# Autodesk Inventor assembly: ASSEMBLY_Main
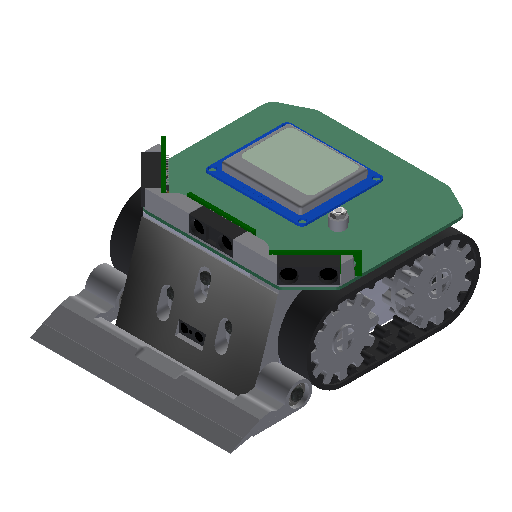
[picture p0: Inventor's stored thumbnail of the model, 512x512]
Saved by Autodesk Inventor 2026.1 (Build 301233000, 233)
## iProperties
Created: 2016-04-29
Part Number: ASSEMBLY_Main
Material: Ogólny
Document SubType Name: Assembly
Designer: Andrzej
Mass: 284.983 g
Surface Area: 1623.62 cm^2
Volume: 252.585 cm^3
Density: 1.12827 g/cm^3
Author: Andrzej
## Documents named in this file (32)
- C:\Users\Andrzej\OneDrive\_DRIVE_SYNCH_FILES\__ BYTECHLAB PROJECTS\MLTDIS - Mini Sumo Robot - Bullet XT\MCAD\1_REV1\ASSEMBLY_MAIN_REVA\ASSEMBLY_Main.iam
- C:\Users\Andrzej\OneDrive\_DRIVE_SYNCH_FILES\__ BYTECHLAB PROJECTS\MLTDIS - Mini Sumo Robot - Bullet XT\MCAD\1_REV1\__COTS_PARTS\COTS_POLOLU_24Dx48L_HP.ipt
- C:\Users\Andrzej\OneDrive\_DRIVE_SYNCH_FILES\__ BYTECHLAB PROJECTS\MLTDIS - Mini Sumo Robot - Bullet XT\MCAD\1_REV1\ASSEMBLY_MAIN_REVA\3DP_PLA_Main_frame.ipt
- C:\Users\Andrzej\OneDrive\_DRIVE_SYNCH_FILES\__ BYTECHLAB PROJECTS\MLTDIS - Mini Sumo Robot - Bullet XT\MCAD\1_REV1\__COTS_PARTS\COTS_AST_604HZZ_Bearing.ipt
- C:\Users\Andrzej\OneDrive\_DRIVE_SYNCH_FILES\__ BYTECHLAB PROJECTS\MLTDIS - Mini Sumo Robot - Bullet XT\MCAD\1_REV1\ASSEMBLY_MAIN_REVA\3DP_PLA_Motor_mounting_bracket_front.ipt
- C:\Users\Andrzej\OneDrive\_DRIVE_SYNCH_FILES\__ BYTECHLAB PROJECTS\MLTDIS - Mini Sumo Robot - Bullet XT\MCAD\1_REV1\__COTS_PARTS\COTS_GENERIC_LiPo_Baterry.ipt
- C:\Users\Andrzej\OneDrive\_DRIVE_SYNCH_FILES\__ BYTECHLAB PROJECTS\MLTDIS - Mini Sumo Robot - Bullet XT\MCAD\1_REV1\__COTS_PARTS\COTS_SHARP_GP2Y0D810Z0F_sensor.ipt
- C:\Users\Andrzej\OneDrive\_DRIVE_SYNCH_FILES\__ BYTECHLAB PROJECTS\MLTDIS - Mini Sumo Robot - Bullet XT\MCAD\1_REV1\ASSEMBLY_MAIN_REVA\3DP_PLA_Front_plow.ipt
- C:\Users\Andrzej\OneDrive\_DRIVE_SYNCH_FILES\__ BYTECHLAB PROJECTS\MLTDIS - Mini Sumo Robot - Bullet XT\MCAD\1_REV1\ASSEMBLY_MAIN_REVA\3DP_PLA_Motor_mounting_bracket_back.ipt
- C:\Users\Andrzej\OneDrive\_DRIVE_SYNCH_FILES\__ BYTECHLAB PROJECTS\MLTDIS - Mini Sumo Robot - Bullet XT\MCAD\1_REV1\__COTS_PARTS\COTS_Nokia_5110_LCD_display.ipt
- C:\Users\Andrzej\OneDrive\_DRIVE_SYNCH_FILES\__ BYTECHLAB PROJECTS\MLTDIS - Mini Sumo Robot - Bullet XT\MCAD\1_REV1\ASSEMBLY_MAIN_REVA\3DP_PLA_Front_motor_clamp_hole_plug.ipt
- C:\Users\Andrzej\OneDrive\_DRIVE_SYNCH_FILES\__ BYTECHLAB PROJECTS\MLTDIS - Mini Sumo Robot - Bullet XT\MCAD\1_REV1\ASSEMBLY_MAIN_REVA\3DP_PLA_Back_motor_clamp_hole_plug.ipt
- C:\Users\Andrzej\OneDrive\_DRIVE_SYNCH_FILES\__ BYTECHLAB PROJECTS\MLTDIS - Mini Sumo Robot - Bullet XT\MCAD\1_REV1\ASSEMBLY_MAIN_REVA\3DP_PLA_Back_slider.ipt
- C:\Users\Andrzej\OneDrive\_DRIVE_SYNCH_FILES\__ BYTECHLAB PROJECTS\MLTDIS - Mini Sumo Robot - Bullet XT\MCAD\1_REV1\ASSEMBLY_MAIN_REVA\ASSEMBLY_PCB_Line_sensor.ipt
- C:\Users\Andrzej\OneDrive\_DRIVE_SYNCH_FILES\__ BYTECHLAB PROJECTS\MLTDIS - Mini Sumo Robot - Bullet XT\MCAD\1_REV1\ASSEMBLY_MAIN_REVA\ASSEMBLY_PCB_Line_sensor_mir.ipt
- C:\Users\Andrzej\OneDrive\_DRIVE_SYNCH_FILES\__ BYTECHLAB PROJECTS\MLTDIS - Mini Sumo Robot - Bullet XT\MCAD\1_REV1\__COTS_PARTS\COTS_SHARP_GP2Y0D810Z0F_sensor_no_pcb.ipt
- C:\Users\Andrzej\OneDrive\_DRIVE_SYNCH_FILES\__ BYTECHLAB PROJECTS\MLTDIS - Mini Sumo Robot - Bullet XT\MCAD\1_REV1\ASSEMBLY_MAIN_REVA\ASSEMBLY_Blade.iam
- C:\Users\Andrzej\OneDrive\_DRIVE_SYNCH_FILES\__ BYTECHLAB PROJECTS\MLTDIS - Mini Sumo Robot - Bullet XT\MCAD\1_REV1\ASSEMBLY_MAIN_REVA\ASSEMBLY_PCB_Motherboard.ipt
- C:\Users\Andrzej\OneDrive\_DRIVE_SYNCH_FILES\__ BYTECHLAB PROJECTS\MLTDIS - Mini Sumo Robot - Bullet XT\MCAD\1_REV1\ASSEMBLY_MAIN_REVA\ASSEMBLY_Tracks.iam
- C:\Users\Andrzej\OneDrive\_DRIVE_SYNCH_FILES\__ BYTECHLAB PROJECTS\MLTDIS - Mini Sumo Robot - Bullet XT\MCAD\1_REV1\__CONTENT_CENTER_PARTS\en-US\ISO 7380-1\ISO 7380-1 - M4 x 25.ipt
- C:\Users\Andrzej\OneDrive\_DRIVE_SYNCH_FILES\__ BYTECHLAB PROJECTS\MLTDIS - Mini Sumo Robot - Bullet XT\MCAD\1_REV1\__CONTENT_CENTER_PARTS\en-US\DIN 125-2  A\DIN 125-2 - A 4,3A.ipt
- C:\Users\Andrzej\OneDrive\_DRIVE_SYNCH_FILES\__ BYTECHLAB PROJECTS\MLTDIS - Mini Sumo Robot - Bullet XT\MCAD\1_REV1\__CONTENT_CENTER_PARTS\en-US\DIN 934\DIN 934 - M4 x 0,7.ipt
- C:\Users\Andrzej\OneDrive\_DRIVE_SYNCH_FILES\__ BYTECHLAB PROJECTS\MLTDIS - Mini Sumo Robot - Bullet XT\MCAD\1_REV1\ASSEMBLY_MAIN_REVA\3DP_PLA_Wheel_cover.ipt
- C:\Users\Andrzej\OneDrive\_DRIVE_SYNCH_FILES\__ BYTECHLAB PROJECTS\MLTDIS - Mini Sumo Robot - Bullet XT\MCAD\1_REV1\__CONTENT_CENTER_PARTS\en-US\ISO 7380-1\ISO 7380-1 - M3 x 30.ipt
- C:\Users\Andrzej\OneDrive\_DRIVE_SYNCH_FILES\__ BYTECHLAB PROJECTS\MLTDIS - Mini Sumo Robot - Bullet XT\MCAD\1_REV1\__CONTENT_CENTER_PARTS\en-US\DIN 934\DIN 934 - M3 x 0,5.ipt
- C:\Users\Andrzej\OneDrive\_DRIVE_SYNCH_FILES\__ BYTECHLAB PROJECTS\MLTDIS - Mini Sumo Robot - Bullet XT\MCAD\1_REV1\__CONTENT_CENTER_PARTS\en-US\DIN 125-2  A\DIN 125-2 - A 3,2A.ipt
- C:\Users\Andrzej\OneDrive\_DRIVE_SYNCH_FILES\__ BYTECHLAB PROJECTS\MLTDIS - Mini Sumo Robot - Bullet XT\MCAD\1_REV1\__CONTENT_CENTER_PARTS\en-US\ISO 7380-1\ISO 7380-1 - M3 x 8.ipt
- C:\Users\Andrzej\OneDrive\_DRIVE_SYNCH_FILES\__ BYTECHLAB PROJECTS\MLTDIS - Mini Sumo Robot - Bullet XT\MCAD\1_REV1\__CONTENT_CENTER_PARTS\en-US\ISO 7380-1\ISO 7380-1 - M3 x 10.ipt
- C:\Users\Andrzej\OneDrive\_DRIVE_SYNCH_FILES\__ BYTECHLAB PROJECTS\MLTDIS - Mini Sumo Robot - Bullet XT\MCAD\1_REV1\__CONTENT_CENTER_PARTS\en-US\ISO 7380-1\ISO 7380-1 - M3 x 25.ipt
- C:\Users\Andrzej\OneDrive\_DRIVE_SYNCH_FILES\__ BYTECHLAB PROJECTS\MLTDIS - Mini Sumo Robot - Bullet XT\MCAD\1_REV1\ASSEMBLY_MAIN_REVA\CUT_M3_Threaded_rod.ipt
- C:\Users\Andrzej\OneDrive\_DRIVE_SYNCH_FILES\__ BYTECHLAB PROJECTS\MLTDIS - Mini Sumo Robot - Bullet XT\MCAD\1_REV1\ASSEMBLY_MAIN_REVA\3DP_PLA_Front_Sharp_sensors_mounting_bracket.ipt
- C:\Users\Andrzej\OneDrive\_DRIVE_SYNCH_FILES\__ BYTECHLAB PROJECTS\MLTDIS - Mini Sumo Robot - Bullet XT\MCAD\1_REV1\ASSEMBLY_MAIN_REVA\3DP_PLA_M3_screw_washer.ipt
## Components (103 placed, 31 different names)
1. COTS_POLOLU_24Dx48L_HP:1 — Równoległy:3, Styczny:7, Styczny:8, Mate:96
2. COTS_POLOLU_24Dx48L_HP:2 — Styczny:1, Równoległy:2, Mate:99
3. 3DP_PLA_Main_frame:1 — Styczny:1, Równoległy:2, Zestawiający:2, Styczny:2, Zestawiający:3, Styczny:3, Zestawiający:4, Styczny:4, Zestawiający:5, Styczny:5, Równoległy:3, Styczny:7, Zestawiający:8, Równoległy:4, Zestawiający:18, Zestawiający:19, Zestawiający:20, Zestawiający:21, Zestawiający:22, Równoległy:6, Równoległy:7, Równoległy:10, Zestawiający:27, Zestawiający:28, Równoległy:11, Równoległy:12, Zestawiający:59, Równoległy:13, Zestawiający:60, Równoległy:14, Równoległy:15, Zestawiający:79, Zestawiający:82, Mate:95, Flush:19, Flush:20, Angle:1, Mate:123, Mate:134, Mate:136, Mate:138, Mate:139, Mate:140, Mate:142, Mate:144, Mate:146, Mate:148, Mate:149, Mate:151, Mate:152, Mate:153, Mate:155, Mate:157, Mate:158, Mate:159, Mate:160, Mate:165, Mate:166, Mate:167, Mate:168
4. COTS_AST_604HZZ_Bearing:1 — Zestawiający:3, Styczny:3, Mate:108
5. COTS_AST_604HZZ_Bearing:2 — Zestawiający:4, Styczny:4, Mate:104
6. COTS_AST_604HZZ_Bearing:3 — Zestawiający:5, Styczny:5, Mate:100
7. COTS_AST_604HZZ_Bearing:4 — Zestawiający:2, Styczny:2, Mate:97, Mate:98
8. 3DP_PLA_Motor_mounting_bracket_front:2 — Zestawiający:8, Styczny:8, Równoległy:4, Zestawiający:57, Mate:125, Mate:127, Mate:129, Mate:131, Mate:141, Mate:143, Mate:145, Mate:147
9. COTS_SHARP_GP2Y0D810Z0F_sensor:1 — Mate:172, Mate:173
10. COTS_SHARP_GP2Y0D810Z0F_sensor:2 — Mate:170, Mate:175
11. COTS_SHARP_GP2Y0D810Z0F_sensor:3 — Mate:171, Mate:174, Mate:176
12. COTS_GENERIC_LiPo_Baterry:1 — Zestawiający:18, Zestawiający:19
13. COTS_GENERIC_LiPo_Baterry:2 — Zestawiający:20, Zestawiający:21
14. 3DP_PLA_Front_plow:1 — Zestawiający:22, Równoległy:6, Równoległy:7, Zestawiający:61, Zestawiający:62, Zestawiający:63, Zestawiający:64, Zestawiający:65, Zestawiający:66, Zestawiający:78, Zestawiający:85, Równoległy:18, Zestawiający:94, Styczny:12, Mate:150, Mate:154, Mate:156
15. 3DP_PLA_Motor_mounting_bracket_back:1 — Równoległy:10, Zestawiający:27, Zestawiający:28, Zestawiający:58, Mate:117, Mate:118, Mate:119, Mate:120, Mate:121, Mate:122, Mate:124, Mate:126, Mate:128, Mate:130, Mate:132, Mate:133, Mate:135, Mate:137
16. COTS_Nokia_5110_LCD_display:1 — Mate:181
17. 3DP_PLA_Front_motor_clamp_hole_plug:1 — Zestawiający:57, Równoległy:11, Równoległy:12
18. 3DP_PLA_Back_motor_clamp_hole_plug:1 — Zestawiający:58, Zestawiający:59, Równoległy:13
19. 3DP_PLA_Back_slider:1 — Zestawiający:60, Równoległy:14, Równoległy:15, Zestawiający:80, Zestawiający:81, Zestawiający:83, Zestawiający:84
20. ASSEMBLY_PCB_Line_sensor:1 — Zestawiający:61, Zestawiający:62, Zestawiający:63
21. ASSEMBLY_PCB_Line_sensor_mir:1 — Zestawiający:64, Zestawiający:65, Zestawiający:66
22. COTS_SHARP_GP2Y0D810Z0F_sensor_no_pcb:1 — Zestawiający:78, Zestawiający:85, Równoległy:18
23. ASSEMBLY_PCB_Line_sensor_mir:2 — Zestawiający:79, Zestawiający:80, Zestawiający:81
24. ASSEMBLY_PCB_Line_sensor:2 — Zestawiający:82, Zestawiający:83, Zestawiający:84
25. ASSEMBLY_Blade:1 [sub-assembly] — Zestawiający:94, Styczny:12, Mate:161, Mate:162, Mate:163, Mate:164
26. ASSEMBLY_PCB_Motherboard:1 — Mate:95, Flush:19, Flush:20, Mate:169, Flush:21, Flush:22, Mate:177, Mate:178, Mate:181
27. ASSEMBLY_Tracks:1 [sub-assembly] — Mate:99, Mate:100, Angle:1, Mate:105, Mate:106, Mate:107, Mate:109, Mate:110, Mate:111, Mate:112
28. ASSEMBLY_Tracks:2 [sub-assembly] — Mate:96, Mate:97, Mate:98, Mate:101, Mate:102, Mate:103, Mate:113, Mate:114, Mate:115, Mate:116
29. 3DP_PLA_Wheel_cover:1 — Mate:110, Mate:111
30. 3DP_PLA_Wheel_cover:2 — Mate:109, Mate:112
31. 3DP_PLA_Wheel_cover:3 — Mate:113, Mate:116
32. 3DP_PLA_Wheel_cover:4 — Mate:114, Mate:115
33. 3DP_PLA_Front_Sharp_sensors_mounting_bracket:1 — Mate:169, Flush:21, Flush:22, Mate:170, Mate:171, Mate:172, Mate:173, Mate:174, Mate:175, Mate:176
34. 3DP_PLA_M3_screw_washer:1 — Mate:177, Mate:180, Insert:38
35. 3DP_PLA_M3_screw_washer:2 — Mate:178, Mate:179, Insert:37
36. ISO 7380-1 M4 x 25:1 — Mate:101, Mate:102
37. DIN 125-2 A A 4,3:1 — Mate:103, Mate:104, Insert:1
38. DIN 934 - replaced by DIN EN 24032/28673/28674 M4:1 — Insert:1
39. ISO 7380-1 M4 x 25:2 — Mate:105, Mate:106
40. DIN 125-2 A A 4,3:2 — Mate:107, Mate:108, Insert:2
41. DIN 934 - replaced by DIN EN 24032/28673/28674 M4:2 — Insert:2
42. DIN 934 - replaced by DIN EN 24032/28673/28674 M3:12 — Insert:37
43. DIN 934 - replaced by DIN EN 24032/28673/28674 M3:13 — Insert:38
44. CUT_M3_Threaded_rod:2 — Mate:166, Mate:168, Mate:180
45. CUT_M3_Threaded_rod:1 — Mate:165, Mate:167, Mate:179
46. ISO 7380-1 M3 x 25:2 — Insert:36
47. DIN 125-2 A A 3,2:34 — Mate:163, Mate:164, Insert:36
48. ISO 7380-1 M3 x 25:1 — Insert:35
49. DIN 125-2 A A 3,2:33 — Mate:161, Mate:162, Insert:35
50. DIN 934 - replaced by DIN EN 24032/28673/28674 M3:11 — Mate:159, Mate:160
51. ISO 7380-1 M3 x 10:2 — Mate:155, Mate:156
52. DIN 934 - replaced by DIN EN 24032/28673/28674 M3:10 — Mate:157, Mate:158
53. ISO 7380-1 M3 x 10:1 — Mate:153, Mate:154
54. DIN 934 - replaced by DIN EN 24032/28673/28674 M3:9 — Mate:151, Mate:152
55. ISO 7380-1 M3 x 8:1 — Mate:149, Mate:150
56. DIN 934 - replaced by DIN EN 24032/28673/28674 M3:8 — Mate:147, Mate:148
57. DIN 934 - replaced by DIN EN 24032/28673/28674 M3:7 — Mate:145, Mate:146
58. DIN 934 - replaced by DIN EN 24032/28673/28674 M3:6 — Mate:143, Mate:144
59. DIN 934 - replaced by DIN EN 24032/28673/28674 M3:5 — Mate:141, Mate:142
60. DIN 934 - replaced by DIN EN 24032/28673/28674 M3:4 — Mate:139, Mate:140
61. DIN 934 - replaced by DIN EN 24032/28673/28674 M3:3 — Mate:137, Mate:138
62. DIN 934 - replaced by DIN EN 24032/28673/28674 M3:2 — Mate:135, Mate:136
63. ISO 7380-1 M3 x 30:8 — Insert:34
64. ISO 7380-1 M3 x 30:7 — Insert:33
65. ISO 7380-1 M3 x 30:6 — Insert:32
66. ISO 7380-1 M3 x 30:5 — Insert:31
67. ISO 7380-1 M3 x 30:4 — Insert:30
68. ISO 7380-1 M3 x 30:3 — Insert:29
69. ISO 7380-1 M3 x 30:2 — Insert:28
70. DIN 125-2 A A 3,2:32 — Insert:26, Insert:34
71. DIN 125-2 A A 3,2:31 — Insert:25, Insert:33
72. DIN 125-2 A A 3,2:30 — Insert:24, Insert:32
73. DIN 125-2 A A 3,2:29 — Insert:23, Insert:31
74. DIN 125-2 A A 3,2:28 — Insert:22, Insert:30
75. DIN 125-2 A A 3,2:27 — Insert:21, Insert:29
76. DIN 125-2 A A 3,2:26 — Insert:20, Insert:28
77. DIN 125-2 A A 3,2:25 — Insert:18, Insert:26
78. DIN 125-2 A A 3,2:24 — Insert:17, Insert:25
79. DIN 125-2 A A 3,2:23 — Insert:16, Insert:24
80. DIN 125-2 A A 3,2:22 — Insert:15, Insert:23
81. DIN 125-2 A A 3,2:21 — Insert:14, Insert:22
82. DIN 125-2 A A 3,2:20 — Insert:13, Insert:21
83. DIN 125-2 A A 3,2:19 — Insert:12, Insert:20
84. DIN 125-2 A A 3,2:18 — Insert:10, Insert:18
85. DIN 125-2 A A 3,2:17 — Insert:9, Insert:17
86. DIN 125-2 A A 3,2:16 — Insert:8, Insert:16
87. DIN 125-2 A A 3,2:15 — Insert:7, Insert:15
88. DIN 125-2 A A 3,2:14 — Insert:6, Insert:14
89. DIN 125-2 A A 3,2:13 — Insert:5, Insert:13
90. DIN 125-2 A A 3,2:12 — Insert:4, Insert:12
91. DIN 125-2 A A 3,2:11 — Mate:131, Mate:132, Insert:10
92. DIN 125-2 A A 3,2:10 — Mate:129, Mate:130, Insert:9
93. DIN 125-2 A A 3,2:9 — Mate:127, Mate:128, Insert:8
94. DIN 125-2 A A 3,2:8 — Mate:125, Mate:126, Insert:7
95. DIN 125-2 A A 3,2:7 — Mate:123, Mate:124, Insert:6
96. DIN 125-2 A A 3,2:6 — Mate:121, Mate:122, Insert:5
97. DIN 125-2 A A 3,2:5 — Mate:119, Mate:120, Insert:4
98. DIN 125-2 A A 3,2:4 — Insert:19, Insert:27
99. DIN 125-2 A A 3,2:3 — Insert:11, Insert:19
100. DIN 125-2 A A 3,2:2 — Insert:3, Insert:11
101. DIN 125-2 A A 3,2:1 — Mate:117, Mate:118, Insert:3
102. DIN 934 - replaced by DIN EN 24032/28673/28674 M3:1 — Mate:133, Mate:134
103. ISO 7380-1 M3 x 30:1 — Insert:27
## Relationships (181: Mate 118, Insert 38, Flush 16, Tangent 8, Angle 1)
- Styczny:1 [Tangent]: COTS_POLOLU_24Dx48L_HP:2 ↔ 3DP_PLA_Main_frame:1
- Równoległy:2 [Flush]: COTS_POLOLU_24Dx48L_HP:2 ↔ 3DP_PLA_Main_frame:1
- Zestawiający:2 [Mate]: 3DP_PLA_Main_frame:1 ↔ COTS_AST_604HZZ_Bearing:4
- Styczny:2 [Tangent]: 3DP_PLA_Main_frame:1 ↔ COTS_AST_604HZZ_Bearing:4
- Zestawiający:3 [Mate]: 3DP_PLA_Main_frame:1 ↔ COTS_AST_604HZZ_Bearing:1
- Styczny:3 [Tangent]: 3DP_PLA_Main_frame:1 ↔ COTS_AST_604HZZ_Bearing:1
- Zestawiający:4 [Mate]: 3DP_PLA_Main_frame:1 ↔ COTS_AST_604HZZ_Bearing:2
- Styczny:4 [Tangent]: 3DP_PLA_Main_frame:1 ↔ COTS_AST_604HZZ_Bearing:2
- Zestawiający:5 [Mate]: 3DP_PLA_Main_frame:1 ↔ COTS_AST_604HZZ_Bearing:3
- Styczny:5 [Tangent]: 3DP_PLA_Main_frame:1 ↔ COTS_AST_604HZZ_Bearing:3
- Równoległy:3 [Flush]: COTS_POLOLU_24Dx48L_HP:1 ↔ 3DP_PLA_Main_frame:1
- Styczny:7 [Tangent]: COTS_POLOLU_24Dx48L_HP:1 ↔ 3DP_PLA_Main_frame:1
- Zestawiający:8 [Mate]: 3DP_PLA_Main_frame:1 ↔ 3DP_PLA_Motor_mounting_bracket_front:2
- Styczny:8 [Tangent]: COTS_POLOLU_24Dx48L_HP:1 ↔ 3DP_PLA_Motor_mounting_bracket_front:2
- Równoległy:4 [Flush]: 3DP_PLA_Main_frame:1 ↔ 3DP_PLA_Motor_mounting_bracket_front:2
- Zestawiający:18 [Mate] (2.5 mm): 3DP_PLA_Main_frame:1 ↔ COTS_GENERIC_LiPo_Baterry:1
- Zestawiający:19 [Mate]: 3DP_PLA_Main_frame:1 ↔ COTS_GENERIC_LiPo_Baterry:1
- Zestawiający:20 [Mate] (2.5 mm): 3DP_PLA_Main_frame:1 ↔ COTS_GENERIC_LiPo_Baterry:2
- Zestawiający:21 [Mate]: 3DP_PLA_Main_frame:1 ↔ COTS_GENERIC_LiPo_Baterry:2
- Zestawiający:22 [Mate]: 3DP_PLA_Main_frame:1 ↔ 3DP_PLA_Front_plow:1
- Równoległy:6 [Flush] (-2 mm): 3DP_PLA_Main_frame:1 ↔ 3DP_PLA_Front_plow:1
- Równoległy:7 [Flush]: 3DP_PLA_Main_frame:1 ↔ 3DP_PLA_Front_plow:1
- Równoległy:10 [Flush]: 3DP_PLA_Main_frame:1 ↔ 3DP_PLA_Motor_mounting_bracket_back:1
- Zestawiający:27 [Mate]: 3DP_PLA_Main_frame:1 ↔ 3DP_PLA_Motor_mounting_bracket_back:1
- Zestawiający:28 [Mate]: 3DP_PLA_Main_frame:1 ↔ 3DP_PLA_Motor_mounting_bracket_back:1
- Zestawiający:57 [Mate]: 3DP_PLA_Motor_mounting_bracket_front:2 ↔ 3DP_PLA_Front_motor_clamp_hole_plug:1
- Równoległy:11 [Flush]: 3DP_PLA_Main_frame:1 ↔ 3DP_PLA_Front_motor_clamp_hole_plug:1
- Równoległy:12 [Flush]: 3DP_PLA_Main_frame:1 ↔ 3DP_PLA_Front_motor_clamp_hole_plug:1
- Zestawiający:58 [Mate]: 3DP_PLA_Motor_mounting_bracket_back:1 ↔ 3DP_PLA_Back_motor_clamp_hole_plug:1
- Zestawiający:59 [Mate]: 3DP_PLA_Main_frame:1 ↔ 3DP_PLA_Back_motor_clamp_hole_plug:1
- Równoległy:13 [Flush]: 3DP_PLA_Main_frame:1 ↔ 3DP_PLA_Back_motor_clamp_hole_plug:1
- Zestawiający:60 [Mate]: 3DP_PLA_Main_frame:1 ↔ 3DP_PLA_Back_slider:1
- Równoległy:14 [Flush]: 3DP_PLA_Main_frame:1 ↔ 3DP_PLA_Back_slider:1
- Równoległy:15 [Flush]: 3DP_PLA_Main_frame:1 ↔ 3DP_PLA_Back_slider:1
- Zestawiający:61 [Mate]: 3DP_PLA_Front_plow:1 ↔ ASSEMBLY_PCB_Line_sensor:1
- Zestawiający:62 [Mate]: 3DP_PLA_Front_plow:1 ↔ ASSEMBLY_PCB_Line_sensor:1
- Zestawiający:63 [Mate]: 3DP_PLA_Front_plow:1 ↔ ASSEMBLY_PCB_Line_sensor:1
- Zestawiający:64 [Mate]: 3DP_PLA_Front_plow:1 ↔ ASSEMBLY_PCB_Line_sensor_mir:1
- Zestawiający:65 [Mate]: 3DP_PLA_Front_plow:1 ↔ ASSEMBLY_PCB_Line_sensor_mir:1
- Zestawiający:66 [Mate]: 3DP_PLA_Front_plow:1 ↔ ASSEMBLY_PCB_Line_sensor_mir:1
- Zestawiający:78 [Mate]: 3DP_PLA_Front_plow:1 ↔ COTS_SHARP_GP2Y0D810Z0F_sensor_no_pcb:1
- Zestawiający:79 [Mate]: 3DP_PLA_Main_frame:1 ↔ ASSEMBLY_PCB_Line_sensor_mir:2
- Zestawiający:80 [Mate]: 3DP_PLA_Back_slider:1 ↔ ASSEMBLY_PCB_Line_sensor_mir:2
- Zestawiający:81 [Mate]: 3DP_PLA_Back_slider:1 ↔ ASSEMBLY_PCB_Line_sensor_mir:2
- Zestawiający:82 [Mate]: 3DP_PLA_Main_frame:1 ↔ ASSEMBLY_PCB_Line_sensor:2
- Zestawiający:83 [Mate]: 3DP_PLA_Back_slider:1 ↔ ASSEMBLY_PCB_Line_sensor:2
- Zestawiający:84 [Mate]: 3DP_PLA_Back_slider:1 ↔ ASSEMBLY_PCB_Line_sensor:2
- Zestawiający:85 [Mate]: 3DP_PLA_Front_plow:1 ↔ COTS_SHARP_GP2Y0D810Z0F_sensor_no_pcb:1
- Równoległy:18 [Flush] (-1 mm): 3DP_PLA_Front_plow:1 ↔ COTS_SHARP_GP2Y0D810Z0F_sensor_no_pcb:1
- Zestawiający:94 [Mate] (1 mm): 3DP_PLA_Front_plow:1 ↔ ASSEMBLY_Blade:1
- Styczny:12 [Tangent]: 3DP_PLA_Front_plow:1 ↔ ASSEMBLY_Blade:1
- Mate:95: 3DP_PLA_Main_frame:1 ↔ ASSEMBLY_PCB_Motherboard:1
- Flush:19: 3DP_PLA_Main_frame:1 ↔ ASSEMBLY_PCB_Motherboard:1
- Flush:20 (-15 mm): 3DP_PLA_Main_frame:1 ↔ ASSEMBLY_PCB_Motherboard:1
- Mate:96: COTS_POLOLU_24Dx48L_HP:1 ↔ ASSEMBLY_Tracks:2
- Mate:97: COTS_AST_604HZZ_Bearing:4 ↔ ASSEMBLY_Tracks:2
- Mate:98: COTS_AST_604HZZ_Bearing:4 ↔ ASSEMBLY_Tracks:2
- Mate:99: COTS_POLOLU_24Dx48L_HP:2 ↔ ASSEMBLY_Tracks:1
- Mate:100: COTS_AST_604HZZ_Bearing:3 ↔ ASSEMBLY_Tracks:1
- Angle:1 (0 deg): 3DP_PLA_Main_frame:1 ↔ ASSEMBLY_Tracks:1
- Mate:101: ASSEMBLY_Tracks:2 ↔ ISO 7380-1 M4 x 25:1
- Mate:102: ASSEMBLY_Tracks:2 ↔ ISO 7380-1 M4 x 25:1
- Mate:103: ASSEMBLY_Tracks:2 ↔ DIN 125-2 A A 4,3:1
- Mate:104: COTS_AST_604HZZ_Bearing:2 ↔ DIN 125-2 A A 4,3:1
- Insert:1: DIN 125-2 A A 4,3:1 ↔ DIN 934 - replaced by DIN EN 24032/28673/28674 M4:1
- Mate:105: ASSEMBLY_Tracks:1 ↔ ISO 7380-1 M4 x 25:2
- Mate:106: ASSEMBLY_Tracks:1 ↔ ISO 7380-1 M4 x 25:2
- Mate:107: ASSEMBLY_Tracks:1 ↔ DIN 125-2 A A 4,3:2
- Mate:108: COTS_AST_604HZZ_Bearing:1 ↔ DIN 125-2 A A 4,3:2
- Insert:2: DIN 125-2 A A 4,3:2 ↔ DIN 934 - replaced by DIN EN 24032/28673/28674 M4:2
- Mate:109: ASSEMBLY_Tracks:1 ↔ 3DP_PLA_Wheel_cover:2
- Mate:110: ASSEMBLY_Tracks:1 ↔ 3DP_PLA_Wheel_cover:1
- Mate:111: ASSEMBLY_Tracks:1 ↔ 3DP_PLA_Wheel_cover:1
- Mate:112: ASSEMBLY_Tracks:1 ↔ 3DP_PLA_Wheel_cover:2
- Mate:113: ASSEMBLY_Tracks:2 ↔ 3DP_PLA_Wheel_cover:3
- Mate:114: ASSEMBLY_Tracks:2 ↔ 3DP_PLA_Wheel_cover:4
- Mate:115: ASSEMBLY_Tracks:2 ↔ 3DP_PLA_Wheel_cover:4
- Mate:116: ASSEMBLY_Tracks:2 ↔ 3DP_PLA_Wheel_cover:3
- Mate:117: 3DP_PLA_Motor_mounting_bracket_back:1 ↔ DIN 125-2 A A 3,2:1
- Mate:118: 3DP_PLA_Motor_mounting_bracket_back:1 ↔ DIN 125-2 A A 3,2:1
- Mate:119: 3DP_PLA_Motor_mounting_bracket_back:1 ↔ DIN 125-2 A A 3,2:5
- Mate:120: 3DP_PLA_Motor_mounting_bracket_back:1 ↔ DIN 125-2 A A 3,2:5
- Mate:121: 3DP_PLA_Motor_mounting_bracket_back:1 ↔ DIN 125-2 A A 3,2:6
- Mate:122: 3DP_PLA_Motor_mounting_bracket_back:1 ↔ DIN 125-2 A A 3,2:6
- Mate:123: 3DP_PLA_Main_frame:1 ↔ DIN 125-2 A A 3,2:7
- Mate:124: 3DP_PLA_Motor_mounting_bracket_back:1 ↔ DIN 125-2 A A 3,2:7
- Mate:125: 3DP_PLA_Motor_mounting_bracket_front:2 ↔ DIN 125-2 A A 3,2:8
- Mate:126: 3DP_PLA_Motor_mounting_bracket_back:1 ↔ DIN 125-2 A A 3,2:8
- Mate:127: 3DP_PLA_Motor_mounting_bracket_front:2 ↔ DIN 125-2 A A 3,2:9
- Mate:128: 3DP_PLA_Motor_mounting_bracket_back:1 ↔ DIN 125-2 A A 3,2:9
- Mate:129: 3DP_PLA_Motor_mounting_bracket_front:2 ↔ DIN 125-2 A A 3,2:10
- Mate:130: 3DP_PLA_Motor_mounting_bracket_back:1 ↔ DIN 125-2 A A 3,2:10
- Mate:131: 3DP_PLA_Motor_mounting_bracket_front:2 ↔ DIN 125-2 A A 3,2:11
- Mate:132: 3DP_PLA_Motor_mounting_bracket_back:1 ↔ DIN 125-2 A A 3,2:11
- Insert:3: DIN 125-2 A A 3,2:2 ↔ DIN 125-2 A A 3,2:1
- Insert:4: DIN 125-2 A A 3,2:12 ↔ DIN 125-2 A A 3,2:5
- Insert:5: DIN 125-2 A A 3,2:13 ↔ DIN 125-2 A A 3,2:6
- Insert:6: DIN 125-2 A A 3,2:14 ↔ DIN 125-2 A A 3,2:7
- Insert:7: DIN 125-2 A A 3,2:15 ↔ DIN 125-2 A A 3,2:8
- Insert:8: DIN 125-2 A A 3,2:16 ↔ DIN 125-2 A A 3,2:9
- Insert:9: DIN 125-2 A A 3,2:17 ↔ DIN 125-2 A A 3,2:10
- Insert:10: DIN 125-2 A A 3,2:18 ↔ DIN 125-2 A A 3,2:11
- Insert:11: DIN 125-2 A A 3,2:3 ↔ DIN 125-2 A A 3,2:2
- Insert:12: DIN 125-2 A A 3,2:19 ↔ DIN 125-2 A A 3,2:12
- Insert:13: DIN 125-2 A A 3,2:20 ↔ DIN 125-2 A A 3,2:13
- Insert:14: DIN 125-2 A A 3,2:21 ↔ DIN 125-2 A A 3,2:14
- Insert:15: DIN 125-2 A A 3,2:22 ↔ DIN 125-2 A A 3,2:15
- Insert:16: DIN 125-2 A A 3,2:23 ↔ DIN 125-2 A A 3,2:16
- Insert:17: DIN 125-2 A A 3,2:24 ↔ DIN 125-2 A A 3,2:17
- Insert:18: DIN 125-2 A A 3,2:25 ↔ DIN 125-2 A A 3,2:18
- Insert:19: DIN 125-2 A A 3,2:4 ↔ DIN 125-2 A A 3,2:3
- Insert:20: DIN 125-2 A A 3,2:26 ↔ DIN 125-2 A A 3,2:19
- Insert:21: DIN 125-2 A A 3,2:27 ↔ DIN 125-2 A A 3,2:20
- Insert:22: DIN 125-2 A A 3,2:28 ↔ DIN 125-2 A A 3,2:21
- Insert:23: DIN 125-2 A A 3,2:29 ↔ DIN 125-2 A A 3,2:22
- Insert:24: DIN 125-2 A A 3,2:30 ↔ DIN 125-2 A A 3,2:23
- Insert:25: DIN 125-2 A A 3,2:31 ↔ DIN 125-2 A A 3,2:24
- Insert:26: DIN 125-2 A A 3,2:32 ↔ DIN 125-2 A A 3,2:25
- Insert:27: DIN 125-2 A A 3,2:4 ↔ ISO 7380-1 M3 x 30:1
- Insert:28: ISO 7380-1 M3 x 30:2 ↔ DIN 125-2 A A 3,2:26
- Insert:29: ISO 7380-1 M3 x 30:3 ↔ DIN 125-2 A A 3,2:27
- Insert:30: ISO 7380-1 M3 x 30:4 ↔ DIN 125-2 A A 3,2:28
- Insert:31: ISO 7380-1 M3 x 30:5 ↔ DIN 125-2 A A 3,2:29
- Insert:32: ISO 7380-1 M3 x 30:6 ↔ DIN 125-2 A A 3,2:30
- Insert:33: ISO 7380-1 M3 x 30:7 ↔ DIN 125-2 A A 3,2:31
- Insert:34: ISO 7380-1 M3 x 30:8 ↔ DIN 125-2 A A 3,2:32
- Mate:133: 3DP_PLA_Motor_mounting_bracket_back:1 ↔ DIN 934 - replaced by DIN EN 24032/28673/28674 M3:1
- Mate:134: 3DP_PLA_Main_frame:1 ↔ DIN 934 - replaced by DIN EN 24032/28673/28674 M3:1
- Mate:135: 3DP_PLA_Motor_mounting_bracket_back:1 ↔ DIN 934 - replaced by DIN EN 24032/28673/28674 M3:2
- Mate:136: 3DP_PLA_Main_frame:1 ↔ DIN 934 - replaced by DIN EN 24032/28673/28674 M3:2
- Mate:137: 3DP_PLA_Motor_mounting_bracket_back:1 ↔ DIN 934 - replaced by DIN EN 24032/28673/28674 M3:3
- Mate:138: 3DP_PLA_Main_frame:1 ↔ DIN 934 - replaced by DIN EN 24032/28673/28674 M3:3
- Mate:139: 3DP_PLA_Main_frame:1 ↔ DIN 934 - replaced by DIN EN 24032/28673/28674 M3:4
- Mate:140: 3DP_PLA_Main_frame:1 ↔ DIN 934 - replaced by DIN EN 24032/28673/28674 M3:4
- Mate:141: 3DP_PLA_Motor_mounting_bracket_front:2 ↔ DIN 934 - replaced by DIN EN 24032/28673/28674 M3:5
- Mate:142: 3DP_PLA_Main_frame:1 ↔ DIN 934 - replaced by DIN EN 24032/28673/28674 M3:5
- Mate:143: 3DP_PLA_Motor_mounting_bracket_front:2 ↔ DIN 934 - replaced by DIN EN 24032/28673/28674 M3:6
- Mate:144: 3DP_PLA_Main_frame:1 ↔ DIN 934 - replaced by DIN EN 24032/28673/28674 M3:6
- Mate:145: 3DP_PLA_Motor_mounting_bracket_front:2 ↔ DIN 934 - replaced by DIN EN 24032/28673/28674 M3:7
- Mate:146: 3DP_PLA_Main_frame:1 ↔ DIN 934 - replaced by DIN EN 24032/28673/28674 M3:7
- Mate:147: 3DP_PLA_Motor_mounting_bracket_front:2 ↔ DIN 934 - replaced by DIN EN 24032/28673/28674 M3:8
- Mate:148: 3DP_PLA_Main_frame:1 ↔ DIN 934 - replaced by DIN EN 24032/28673/28674 M3:8
- Mate:149: 3DP_PLA_Main_frame:1 ↔ ISO 7380-1 M3 x 8:1
- Mate:150: 3DP_PLA_Front_plow:1 ↔ ISO 7380-1 M3 x 8:1
- Mate:151: 3DP_PLA_Main_frame:1 ↔ DIN 934 - replaced by DIN EN 24032/28673/28674 M3:9
- Mate:152: 3DP_PLA_Main_frame:1 ↔ DIN 934 - replaced by DIN EN 24032/28673/28674 M3:9
- Mate:153: 3DP_PLA_Main_frame:1 ↔ ISO 7380-1 M3 x 10:1
- Mate:154: 3DP_PLA_Front_plow:1 ↔ ISO 7380-1 M3 x 10:1
- Mate:155: 3DP_PLA_Main_frame:1 ↔ ISO 7380-1 M3 x 10:2
- Mate:156: 3DP_PLA_Front_plow:1 ↔ ISO 7380-1 M3 x 10:2
- Mate:157: 3DP_PLA_Main_frame:1 ↔ DIN 934 - replaced by DIN EN 24032/28673/28674 M3:10
- Mate:158: 3DP_PLA_Main_frame:1 ↔ DIN 934 - replaced by DIN EN 24032/28673/28674 M3:10
- Mate:159: 3DP_PLA_Main_frame:1 ↔ DIN 934 - replaced by DIN EN 24032/28673/28674 M3:11
- Mate:160: 3DP_PLA_Main_frame:1 ↔ DIN 934 - replaced by DIN EN 24032/28673/28674 M3:11
- Mate:161: ASSEMBLY_Blade:1 ↔ DIN 125-2 A A 3,2:33
- Mate:162: ASSEMBLY_Blade:1 ↔ DIN 125-2 A A 3,2:33
- Insert:35: ISO 7380-1 M3 x 25:1 ↔ DIN 125-2 A A 3,2:33
- Mate:163: ASSEMBLY_Blade:1 ↔ DIN 125-2 A A 3,2:34
- Mate:164: ASSEMBLY_Blade:1 ↔ DIN 125-2 A A 3,2:34
- Insert:36: ISO 7380-1 M3 x 25:2 ↔ DIN 125-2 A A 3,2:34
- Mate:165: 3DP_PLA_Main_frame:1 ↔ CUT_M3_Threaded_rod:1
- Mate:166: 3DP_PLA_Main_frame:1 ↔ CUT_M3_Threaded_rod:2
- Mate:167 (5 mm): 3DP_PLA_Main_frame:1 ↔ CUT_M3_Threaded_rod:1
- Mate:168 (5 mm): 3DP_PLA_Main_frame:1 ↔ CUT_M3_Threaded_rod:2
- Mate:169: ASSEMBLY_PCB_Motherboard:1 ↔ 3DP_PLA_Front_Sharp_sensors_mounting_bracket:1
- Flush:21: ASSEMBLY_PCB_Motherboard:1 ↔ 3DP_PLA_Front_Sharp_sensors_mounting_bracket:1
- Flush:22: ASSEMBLY_PCB_Motherboard:1 ↔ 3DP_PLA_Front_Sharp_sensors_mounting_bracket:1
- Mate:170: COTS_SHARP_GP2Y0D810Z0F_sensor:2 ↔ 3DP_PLA_Front_Sharp_sensors_mounting_bracket:1
- Mate:171: COTS_SHARP_GP2Y0D810Z0F_sensor:3 ↔ 3DP_PLA_Front_Sharp_sensors_mounting_bracket:1
- Mate:172: COTS_SHARP_GP2Y0D810Z0F_sensor:1 ↔ 3DP_PLA_Front_Sharp_sensors_mounting_bracket:1
- Mate:173: COTS_SHARP_GP2Y0D810Z0F_sensor:1 ↔ 3DP_PLA_Front_Sharp_sensors_mounting_bracket:1
- Mate:174: COTS_SHARP_GP2Y0D810Z0F_sensor:3 ↔ 3DP_PLA_Front_Sharp_sensors_mounting_bracket:1
- Mate:175: COTS_SHARP_GP2Y0D810Z0F_sensor:2 ↔ 3DP_PLA_Front_Sharp_sensors_mounting_bracket:1
- Mate:176: COTS_SHARP_GP2Y0D810Z0F_sensor:3 ↔ 3DP_PLA_Front_Sharp_sensors_mounting_bracket:1
- Mate:177: ASSEMBLY_PCB_Motherboard:1 ↔ 3DP_PLA_M3_screw_washer:1
- Mate:178: ASSEMBLY_PCB_Motherboard:1 ↔ 3DP_PLA_M3_screw_washer:2
- Mate:179: 3DP_PLA_M3_screw_washer:2 ↔ CUT_M3_Threaded_rod:1
- Mate:180: 3DP_PLA_M3_screw_washer:1 ↔ CUT_M3_Threaded_rod:2
- Insert:37: 3DP_PLA_M3_screw_washer:2 ↔ DIN 934 - replaced by DIN EN 24032/28673/28674 M3:12
- Insert:38: 3DP_PLA_M3_screw_washer:1 ↔ DIN 934 - replaced by DIN EN 24032/28673/28674 M3:13
- Mate:181 (10 mm): COTS_Nokia_5110_LCD_display:1 ↔ ASSEMBLY_PCB_Motherboard:1
